# Autodesk Inventor assembly: MX-64T
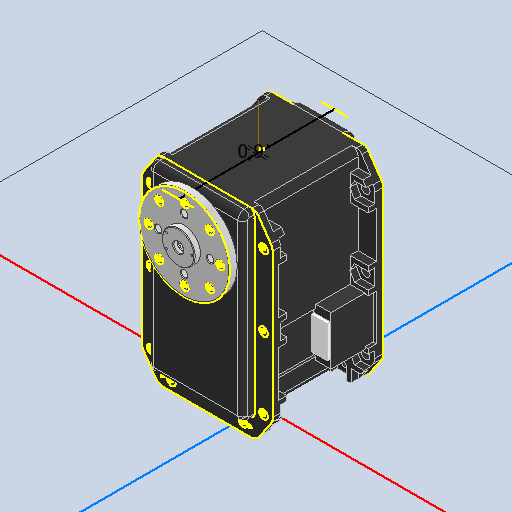
[picture p0: Inventor's stored thumbnail of the model, 512x512]
Saved by Autodesk Inventor 2022 (Build 260153000, 153)
## iProperties
Created: 2022-11-17
Part Number: MX-64T
Document SubType Name: Assembly
Designer: Petrov Ivan
Mass: 72.06 g
Surface Area: 159.232 cm^2
Volume: 72.06 cm^3
Density: 1 g/cm^3
Author: Petrov Ivan
## Documents named in this file (3)
- C:\Users\Ivan Petrov\Documents\GitHub\OmniBot\design\standart_components\dynamixels\mx-64\MX-64T.iam
- C:\Users\Ivan Petrov\Documents\GitHub\OmniBot\design\standart_components\dynamixels\mx-64\MX-64T.ipt
- C:\Users\Ivan Petrov\Documents\GitHub\OmniBot\design\standart_components\dynamixels\mx-64\HN05-N101.ipt
## Components (2 placed, 2 different names)
1. MX-64T:1 — Совмещение:1, Совмещение:2
2. HN05-N101:1 — Совмещение:1, Совмещение:2
## Relationships (2: Mate 2)
- Совмещение:1 [Mate]: MX-64T:1 ↔ HN05-N101:1
- Совмещение:2 [Mate]: MX-64T:1 ↔ HN05-N101:1
